# Autodesk Inventor assembly: Rly Cool 4 in Traction Wheel
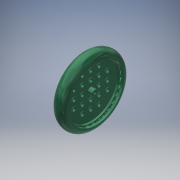
[picture p0: Inventor's stored thumbnail of the model, 180x180]
Saved by Autodesk Inventor 2019 (Build 230136000, 136)
## iProperties
Created: 2020-04-29
Part Number: Rly Cool 4 in Traction Wheel
Document SubType Name: Assembly
Designer: karlv
Author: karlv
## Documents named in this file (3)
- C:\Users\karlv\Documents\VEX\62019S Repos\2020-2021_CAD\Karl CAD Lib\Wheels\Rly Cool 4 in Traction Wheel.iam
- C:\Users\karlv\Documents\VEX\62019S Repos\2020-2021_CAD\Karl CAD Lib\Sprockets\HS\30T HS Sprocket (LS Bore).ipt
- C:\Users\karlv\Documents\VEX\62019S Repos\2020-2021_CAD\Karl CAD Lib\Wheels\4_High_Traction_Tire_276-1489.ipt
## Components (2 placed, 2 different names)
1. 30T HS Sprocket (LS Bore):1 — Mate:1, Mate:2
2. 4_High_Traction_Tire_276-1489:1 — Mate:1, Mate:2
## Relationships (2: Mate 2)
- Mate:1 (2.4511 mm): 30T HS Sprocket (LS Bore):1 ↔ 4_High_Traction_Tire_276-1489:1
- Mate:2: 30T HS Sprocket (LS Bore):1 ↔ 4_High_Traction_Tire_276-1489:1
